# Autodesk Inventor assembly: 6 bar_MIR
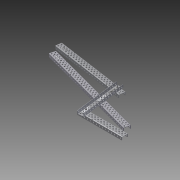
[picture p0: Inventor's stored thumbnail of the model, 180x180]
Saved by Autodesk Inventor 2014 (Build 180170000, 170)
## iProperties
Created: 2013-09-14
Part Number: 6 bar_MIR
Document SubType Name: Assembly
Designer: Ryan
Author: Ryan
## Documents named in this file (8)
- C:\Users\Ryan\Desktop\sw\6 bar\6 bar_MIR.iam
- C:\Users\Ryan\Desktop\sw\lib\Aperture VEX CAD Library\Metal\C Channel\2 x 35.ipt
- C:\Users\Ryan\Desktop\sw\lib\Aperture VEX CAD Library\Metal\C Channel\2 x 25.ipt
- C:\Users\Ryan\Desktop\sw\lib\Aperture VEX CAD Library\Metal\C Channel\2 x 15.ipt
- C:\Users\Ryan\Desktop\sw\lib\Aperture VEX CAD Library\Bearing Blocks\Bearing Block.ipt
- C:\Users\Ryan\Desktop\sw\lib\Aperture VEX CAD Library\Spacers\SPACER-0500-0125.ipt
- C:\Users\Ryan\Desktop\sw\lib\Aperture VEX CAD Library\Hardware\8-32\8-32_.375.ipt
- C:\Users\Ryan\Desktop\sw\lib\Aperture VEX CAD Library\Hardware\8-32\8-32_.875.ipt
## Components (37 placed, 7 different names)
1. 2 x 35:1 — Angle:1, Mate:39, Mate:42, Mate:41, Mate:40, Mate:45, Mate:82, Mate:80, Mate:79, Mate:87, Mate:81, Mate:72, Mate:73, Mate:74, Mate:75, Mate:78, Mate:79
2. 2 x 25:1 — Angle:1, Mate:50, Mate:52, Mate:51, Mate:53, Mate:60, Mate:70, Mate:71, Mate:82, Mate:83, Mate:84, Mate:85, Mate:86, Mate:87
3. 2 x 15:1 — Mate:1, Mate:10, Mate:15, Mate:12, Mate:14, Mate:83, Mate:17, Mate:16
4. Bearing Block:1 — Mate:1, Mate:9, Mate:11, Mate:13, Mate:26, Mate:64
5. 2 x 15:2 — Mate:27, Mate:20, Mate:24, Mate:23, Mate:21, Mate:86, Mate:85, Mate:84, Mate:25, Mate:22, Mate:30, Mate:56, Mate:34, Mate:32, Mate:44, Mate:62, Mate:57, Mate:54, Mate:59
6. SPACER-0500-0125:1 — Mate:27, Mate:10, Mate:9
7. 8-32_.375:1 — Mate:15, Mate:12, Mate:11, Mate:16
8. 8-32_.375:2 — Mate:14, Mate:13, Mate:83, Mate:17
9. Bearing Block:3 — Mate:30, Mate:28, Mate:58, Mate:55
10. 8-32_.375:5 — Mate:56, Mate:34, Mate:32, Mate:28
11. Bearing Block:4 — Mate:39, Mate:36, Mate:38, Mate:37, Mate:46, Mate:67, Mate:65, Mate:43
12. 8-32_.375:6 — Mate:42, Mate:36, Flush:1
13. 8-32_.375:7 — Mate:41, Mate:40, Flush:1, Mate:38, Mate:37
14. SPACER-0500-0125:2 — Mate:46, Mate:45, Mate:44
15. Bearing Block:5 — Mate:58, Mate:50, Mate:47, Mate:48, Mate:49, Mate:61, Mate:68, Mate:66
16. 8-32_.375:8 — Mate:52, Mate:51, Mate:47, Flush:2, Mate:71
17. 8-32_.375:9 — Mate:53, Mate:48, Flush:2, Mate:49, Mate:70
18. 8-32_.375:10 — Mate:62, Mate:57, Mate:55, Mate:54
19. SPACER-0500-0125:3 — Mate:61, Mate:60, Mate:59
20. 8-32_.875:1 — Mate:64, Mate:63
21. 8-32_.875:2 — Mate:68, Mate:66
22. 8-32_.875:3 — Mate:67, Mate:65
23. Bearing Block:6 — Mate:82, Mate:76, Mate:77, Mate:78
24. 8-32_.375:11 — Mate:80, Mate:79, Mate:76, Flush:4
25. 8-32_.375:12 — Mate:87, Mate:81, Mate:77, Flush:4, Mate:78
26. Bearing Block:8 — Mate:72, Mate:73, Mate:74, Mate:75, Mate:76, Mate:77
27. 8-32_.375:15 — Mate:81, Mate:84
28. 8-32_.375:16 — Mate:80, Mate:83, Mate:87
29. 8-32_.375:17 — Mate:77, Mate:78
30. 8-32_.375:18 — Mate:76, Mate:79
31. Bearing Block:9 — Mate:80, Mate:81, Mate:82, Mate:85, Mate:86
32. 8-32_.375:4 — Mate:86, Mate:85, Mate:84, Mate:25, Mate:22, Mate:19
33. Bearing Block:2 — Mate:26, Mate:20, Mate:18, Mate:19, Mate:63
34. 8-32_.375:3 — Mate:24, Mate:23, Mate:21, Mate:18
35. 8-32_.375:13
36. Bearing Block:7 — Mate:43
37. 8-32_.375:14
## Component patterns: (2 elements, first: 8-32_.375:4 + Bearing Block:2 + 8-32_.375:3)
## Relationships (91: Mate 87, Flush 3, Angle 1)
- Angle:1 (180 deg): 2 x 35:1 ↔ 2 x 25:1
- Mate:1: 2 x 15:1 ↔ Bearing Block:1
- Mate:27: 2 x 15:2 ↔ SPACER-0500-0125:1
- Mate:10: 2 x 15:1 ↔ SPACER-0500-0125:1
- Mate:9: Bearing Block:1 ↔ SPACER-0500-0125:1
- Mate:15 (2.3114 mm): 2 x 15:1 ↔ 8-32_.375:1
- Mate:12: 2 x 15:1 ↔ 8-32_.375:1
- Mate:11: Bearing Block:1 ↔ 8-32_.375:1
- Mate:14: 2 x 15:1 ↔ 8-32_.375:2
- Mate:13: Bearing Block:1 ↔ 8-32_.375:2
- Mate:83 (2.3114 mm): 2 x 15:1 ↔ 8-32_.375:2
- Mate:17 (2.3114 mm): 2 x 15:1 ↔ 8-32_.375:2
- Mate:16 (2.3114 mm): 2 x 15:1 ↔ 8-32_.375:1
- Mate:26: Bearing Block:1 ↔ Bearing Block:2
- Mate:20: 2 x 15:2 ↔ Bearing Block:2
- Mate:24 (2.3114 mm): 2 x 15:2 ↔ 8-32_.375:3
- Mate:23 (2.3114 mm): 2 x 15:2 ↔ 8-32_.375:3
- Mate:21: 2 x 15:2 ↔ 8-32_.375:3
- Mate:18: Bearing Block:2 ↔ 8-32_.375:3
- Mate:86 (2.3114 mm): 2 x 15:2 ↔ 8-32_.375:4
- Mate:85 (2.3114 mm): 2 x 15:2 ↔ 8-32_.375:4
- Mate:84 (2.3114 mm): 2 x 15:2 ↔ 8-32_.375:4
- Mate:25 (2.3114 mm): 2 x 15:2 ↔ 8-32_.375:4
- Mate:22: 2 x 15:2 ↔ 8-32_.375:4
- Mate:19: 8-32_.375:4 ↔ Bearing Block:2
- Mate:30: 2 x 15:2 ↔ Bearing Block:3
- Mate:56 (2.3114 mm): 2 x 15:2 ↔ 8-32_.375:5
- Mate:34 (2.3114 mm): 2 x 15:2 ↔ 8-32_.375:5
- Mate:32: 2 x 15:2 ↔ 8-32_.375:5
- Mate:28: Bearing Block:3 ↔ 8-32_.375:5
- Mate:39: 2 x 35:1 ↔ Bearing Block:4
- Mate:42 (2.3114 mm): 2 x 35:1 ↔ 8-32_.375:6
- Mate:36: Bearing Block:4 ↔ 8-32_.375:6
- Mate:41 (2.3114 mm): 2 x 35:1 ↔ 8-32_.375:7
- Mate:40 (2.3114 mm): 2 x 35:1 ↔ 8-32_.375:7
- Flush:1: 8-32_.375:6 ↔ 8-32_.375:7
- Mate:38 (1.1684 mm): Bearing Block:4 ↔ 8-32_.375:7
- Mate:37: Bearing Block:4 ↔ 8-32_.375:7
- Mate:46: Bearing Block:4 ↔ SPACER-0500-0125:2
- Mate:45: 2 x 35:1 ↔ SPACER-0500-0125:2
- Mate:44: 2 x 15:2 ↔ SPACER-0500-0125:2
- Mate:58: Bearing Block:3 ↔ Bearing Block:5
- Mate:50: 2 x 25:1 ↔ Bearing Block:5
- Mate:52 (2.3114 mm): 2 x 25:1 ↔ 8-32_.375:8
- Mate:51 (2.3114 mm): 2 x 25:1 ↔ 8-32_.375:8
- Mate:47: Bearing Block:5 ↔ 8-32_.375:8
- Mate:53 (2.3114 mm): 2 x 25:1 ↔ 8-32_.375:9
- Mate:48: Bearing Block:5 ↔ 8-32_.375:9
- Flush:2: 8-32_.375:8 ↔ 8-32_.375:9
- Mate:49 (1.1684 mm): Bearing Block:5 ↔ 8-32_.375:9
- Mate:62 (2.3114 mm): 2 x 15:2 ↔ 8-32_.375:10
- Mate:57 (2.3114 mm): 2 x 15:2 ↔ 8-32_.375:10
- Mate:55: Bearing Block:3 ↔ 8-32_.375:10
- Mate:54: 2 x 15:2 ↔ 8-32_.375:10
- Mate:61: Bearing Block:5 ↔ SPACER-0500-0125:3
- Mate:60: 2 x 25:1 ↔ SPACER-0500-0125:3
- Mate:59: 2 x 15:2 ↔ SPACER-0500-0125:3
- Mate:64: Bearing Block:1 ↔ 8-32_.875:1
- Mate:63: 8-32_.875:1 ↔ Bearing Block:2
- Mate:68: Bearing Block:5 ↔ 8-32_.875:2
- Mate:66: Bearing Block:5 ↔ 8-32_.875:2
- Mate:67: Bearing Block:4 ↔ 8-32_.875:3
- Mate:65: Bearing Block:4 ↔ 8-32_.875:3
- Mate:82: 2 x 35:1 ↔ Bearing Block:6
- Mate:80 (2.3114 mm): 2 x 35:1 ↔ 8-32_.375:11
- Mate:79 (2.3114 mm): 2 x 35:1 ↔ 8-32_.375:11
- Mate:76: Bearing Block:6 ↔ 8-32_.375:11
- Mate:87 (2.3114 mm): 2 x 35:1 ↔ 8-32_.375:12
- Mate:81 (2.3114 mm): 2 x 35:1 ↔ 8-32_.375:12
- Mate:77: Bearing Block:6 ↔ 8-32_.375:12
- Flush:4: 8-32_.375:11 ↔ 8-32_.375:12
- Mate:78 (1.1684 mm): Bearing Block:6 ↔ 8-32_.375:12
- Mate:43: Bearing Block:4 ↔ Bearing Block:7
- Mate:70 (2.3114 mm): 2 x 25:1 ↔ 8-32_.375:9
- Mate:71 (2.3114 mm): 2 x 25:1 ↔ 8-32_.375:8
- Mate:72: 2 x 35:1 ↔ Bearing Block:8
- Mate:73 (2.3114 mm): 2 x 35:1 ↔ Bearing Block:8
- Mate:74 (2.3114 mm): 2 x 35:1 ↔ Bearing Block:8
- Mate:75 (2.3114 mm): 2 x 35:1 ↔ Bearing Block:8
- Mate:76: Bearing Block:8 ↔ 8-32_.375:18
- Mate:77: Bearing Block:8 ↔ 8-32_.375:17
- Mate:78: 2 x 35:1 ↔ 8-32_.375:17
- Mate:79: 2 x 35:1 ↔ 8-32_.375:18
- Mate:80: 8-32_.375:16 ↔ Bearing Block:9
- Mate:81: 8-32_.375:15 ↔ Bearing Block:9
- Mate:82: 2 x 25:1 ↔ Bearing Block:9
- Mate:83: 2 x 25:1 ↔ 8-32_.375:16
- Mate:84: 2 x 25:1 ↔ 8-32_.375:15
- Mate:85 (2.3114 mm): 2 x 25:1 ↔ Bearing Block:9
- Mate:86 (2.3114 mm): 2 x 25:1 ↔ Bearing Block:9
- Mate:87 (2.3114 mm): 2 x 25:1 ↔ 8-32_.375:16
## Named parameters: q = 2.3114 mm
